# Autodesk Inventor assembly: DIFF_BARV2_ASM
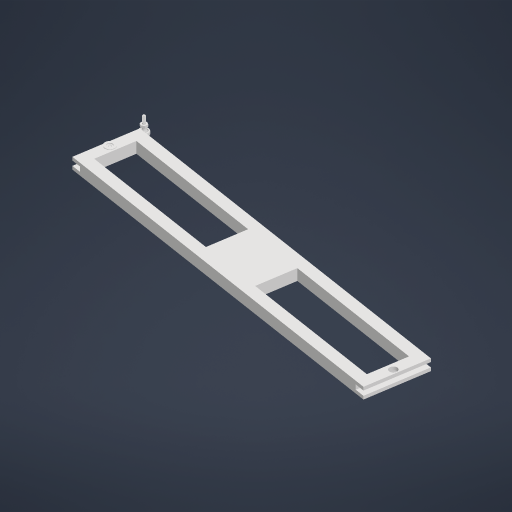
[picture p0: Inventor's stored thumbnail of the model, 512x512]
Saved by Autodesk Inventor 2023 (Build 270158000, 158)
## iProperties
Created: 2023-04-06
Part Number: DIFF_BARV2_ASM
Document SubType Name: Assembly
Designer: bugme
Author: bugme
## Documents named in this file (6)
- C:\Users\bugme\Desktop\Diff Bar\DIFF_BARV2_ASM.iam
- C:\Users\bugme\Desktop\Diff Bar\Diff_BarV2.ipt
- C:\Users\bugme\Desktop\Diff Bar\60645K211_Ball Joint Linkage.ipt
- C:\Users\bugme\Desktop\Diff Bar\59915K481_Corrosion-Resistant Ball Joint Rod End.ipt
- C:\Users\bugme\Desktop\Diff Bar\98381A505_Dowel Pin.ipt
- C:\Users\bugme\Desktop\Diff Bar\1293N114_Self-Aligning Flanged Ball Bearing.ipt
## Components (5 placed, 5 different names)
1. Diff_BarV2:1 — Insert:1
2. 60645K211_Ball Joint Linkage:1 — Insert:4
3. 59915K481_Corrosion-Resistant Ball Joint Rod End:1 — Insert:3, Insert:4
4. 98381A505_Dowel Pin:1 — Insert:2, Insert:3
5. 1293N114_Self-Aligning Flanged Ball Bearing:1 — Insert:1, Insert:2
## Relationships (4: Insert 4)
- Insert:1: Diff_BarV2:1 ↔ 1293N114_Self-Aligning Flanged Ball Bearing:1
- Insert:2: 98381A505_Dowel Pin:1 ↔ 1293N114_Self-Aligning Flanged Ball Bearing:1
- Insert:3: 59915K481_Corrosion-Resistant Ball Joint Rod End:1 ↔ 98381A505_Dowel Pin:1
- Insert:4: 60645K211_Ball Joint Linkage:1 ↔ 59915K481_Corrosion-Resistant Ball Joint Rod End:1
